# Autodesk Inventor assembly: Frame 1771926384246
(part 3 of 3)
212. ANSI UP8 x 30 - 125.591:133
213. ANSI UP8 x 30 - 125.591:134
214. ANSI UP8 x 30 - 125.591:135
215. ANSI UP8 x 30 - 81.102:79
216. ANSI UP8 x 30 - 125.591:136
217. ANSI UP8 x 30 - 125.591:137
218. ANSI UP8 x 30 - 125.591:138
219. ANSI UP8 x 30 - 81.102:80
220. ANSI UP8 x 30 - 125.591:139
221. ANSI UP8 x 30 - 125.591:140
222. ANSI UP8 x 30 - 81.102:81
223. ANSI UP8 x 30 - 125.591:141
224. ANSI UP8 x 30 - 125.591:142
225. ANSI UP8 x 30 - 81.102:82
226. ANSI UP8 x 30 - 125.591:143
227. ANSI UP8 x 30 - 81.102:83
228. ANSI UP8 x 30 - 125.591:144
229. ANSI UP8 x 30 - 125.591:145
230. ANSI UP8 x 30 - 125.591:146
231. ANSI UP8 x 30 - 125.591:147
232. ANSI UP8 x 30 - 81.102:84
233. ANSI UP8 x 30 - 125.591:148
234. ANSI UP8 x 30 - 125.591:149
235. ANSI UP8 x 30 - 81.102:85
236. ANSI UP8 x 30 - 81.102:86
237. ANSI UP8 x 30 - 125.591:150
238. ANSI UP8 x 30 - 125.591:151
239. ANSI UP8 x 30 - 81.102:87
240. ANSI UP8 x 30 - 125.591:152
241. ANSI UP8 x 30 - 81.102:88
242. ANSI UP8 x 30 - 125.591:153
243. ANSI UP8 x 30 - 81.102:89
244. ANSI UP8 x 30 - 125.591:154
245. ANSI UP8 x 30 - 81.102:90
246. ANSI UP8 x 30 - 125.591:155
247. ANSI UP8 x 30 - 81.102:91
248. ANSI UP8 x 30 - 81.102:92
249. ANSI UP8 x 30 - 125.591:156
250. ANSI UP8 x 30 - 125.591:157
251. ANSI UP8 x 30 - 81.102:93
252. ANSI UP8 x 30 - 81.102:94
253. ANSI UP8 x 30 - 125.591:158
254. ANSI UP8 x 30 - 125.591:159
255. ANSI UP8 x 30 - 81.102:95
256. ANSI UP8 x 30 - 81.102:96
257. ANSI UP8 x 30 - 125.591:160
258. ANSI UP8 x 30 - 125.591:161
259. ANSI UP8 x 30 - 81.102:97
260. ANSI UP8 x 30 - 81.102:98
261. ANSI UP8 x 30 - 125.591:162
262. ANSI UP8 x 30 - 125.591:163
263. ANSI UP8 x 30 - 125.591:164
264. ANSI UP8 x 30 - 125.591:165
265. ANSI UP8 x 30 - 125.591:166
266. ANSI UP8 x 30 - 125.591:167
267. ANSI UP8 x 30 - 125.591:168
268. ANSI UP8 x 30 - 125.591:169
269. ANSI UP8 x 30 - 125.591:170
270. ANSI UP8 x 30 - 125.591:171
271. ANSI UP8 x 30 - 125.591:172
272. ANSI UP8 x 30 - 125.591:173
273. ANSI UP8 x 30 - 125.591:174
274. ANSI UP8 x 30 - 125.591:175
275. ANSI UP8 x 30 - 81.102:99
276. ANSI UP8 x 30 - 81.102:100
277. ANSI UP8 x 30 - 125.591:176
278. ANSI UP8 x 30 - 125.591:177
279. ANSI UP8 x 30 - 125.591:178
280. ANSI UP8 x 30 - 125.591:179
281. ANSI UP8 x 30 - 81.102:101
282. ANSI UP8 x 30 - 125.591:180
283. ANSI UP8 x 30 - 125.591:181
284. ANSI UP8 x 30 - 81.102:102
285. ANSI UP8 x 30 - 125.591:182
286. ANSI UP8 x 30 - 125.591:183
287. ANSI UP8 x 30 - 81.102:103
288. ANSI UP8 x 30 - 125.591:184
289. ANSI UP8 x 30 - 81.102:104
290. ANSI UP8 x 30 - 125.591:185
291. ANSI UP8 x 30 - 125.591:186
292. ANSI UP8 x 30 - 81.102:105
293. ANSI UP8 x 30 - 125.591:187
294. ANSI UP8 x 30 - 125.591:188
295. ANSI UP8 x 30 - 81.102:106
296. ANSI UP8 x 30 - 125.591:189
297. ANSI UP8 x 30 - 81.102:107
298. ANSI UP8 x 30 - 125.591:190
299. ANSI UP8 x 30 - 81.102:108
300. ANSI UP8 x 30 - 125.591:191
301. ANSI UP8 x 30 - 81.102:109
302. ANSI UP8 x 30 - 125.591:192
303. ANSI UP8 x 30 - 81.102:110
304. ANSI UP8 x 30 - 125.591:193
305. ANSI UP8 x 30 - 81.102:111
306. ANSI UP8 x 30 - 125.591:194
307. ANSI UP8 x 30 - 81.102:112
308. ANSI UP8 x 30 - 125.591:195
309. ANSI UP8 x 30 - 81.102:113
310. ANSI UP8 x 30 - 125.591:196
311. ANSI UP8 x 30 - 81.102:114
312. ANSI UP8 x 30 - 125.591:197
313. ANSI UP8 x 30 - 81.102:115
314. ANSI UP8 x 30 - 81.102:116
315. ANSI UP8 x 30 - 125.591:198
316. ANSI UP8 x 30 - 125.591:199
317. ANSI UP8 x 30 - 81.102:117
318. ANSI UP8 x 30 - 81.102:118
319. ANSI UP8 x 30 - 125.591:200
320. ANSI UP8 x 30 - 125.591:201
321. ANSI UP8 x 30 - 81.102:119
322. ANSI UP8 x 30 - 81.102:120
323. ANSI UP8 x 30 - 125.591:202
324. ANSI UP8 x 30 - 125.591:203
325. ANSI UP8 x 30 - 125.591:204
326. ANSI UP8 x 30 - 125.591:205
327. ANSI UP8 x 30 - 125.591:206
328. ANSI UP8 x 30 - 125.591:207
329. ANSI UP8 x 30 - 125.591:208
330. ANSI UP8 x 30 - 125.591:209
331. ANSI UP8 x 30 - 125.591:210
332. ANSI UP8 x 30 - 125.591:211
333. ANSI UP8 x 30 - 125.591:212
334. ANSI UP8 x 30 - 125.591:213
335. ANSI UP8 x 30 - 125.591:214
336. ANSI UP8 x 30 - 125.591:215
337. ANSI UP8 x 30 - 125.591:216
338. ANSI UP8 x 30 - 81.102:121
339. ANSI UP8 x 30 - 125.591:217
340. ANSI UP8 x 30 - 125.591:218
341. ANSI UP8 x 30 - 81.102:122
342. ANSI UP8 x 30 - 125.591:219
343. ANSI UP8 x 30 - 125.591:220
344. ANSI UP8 x 30 - 81.102:123
345. ANSI UP8 x 30 - 81.102:124
346. ANSI UP8 x 30 - 125.591:221
347. ANSI UP8 x 30 - 125.591:222
348. ANSI UP8 x 30 - 125.591:223
349. ANSI UP8 x 30 - 125.591:224
350. ANSI UP8 x 30 - 81.102:125
351. ANSI UP8 x 30 - 125.591:225
352. ANSI UP8 x 30 - 125.591:226
353. ANSI UP8 x 30 - 81.102:126
354. ANSI UP8 x 30 - 125.591:227
355. ANSI UP8 x 30 - 125.591:228
356. ANSI UP8 x 30 - 125.591:229
357. ANSI UP8 x 30 - 125.591:230
358. ANSI UP8 x 30 - 81.102:127
359. ANSI UP8 x 30 - 81.102:128
360. ANSI UP8 x 30 - 125.591:231
361. ANSI UP8 x 30 - 81.102:129
362. ANSI UP8 x 30 - 125.591:232
363. ANSI UP8 x 30 - 81.102:130
364. ANSI UP8 x 30 - 81.102:131
365. ANSI UP8 x 30 - 125.591:233
366. ANSI UP8 x 30 - 125.591:234
367. ANSI UP8 x 30 - 81.102:132
368. ANSI UP8 x 30 - 125.591:235
369. ANSI UP8 x 30 - 125.591:236
370. ANSI UP8 x 30 - 81.102:133
371. ANSI UP8 x 30 - 81.102:134
372. ANSI UP8 x 30 - 125.591:237
373. ANSI UP8 x 30 - 81.102:135
374. ANSI UP8 x 30 - 125.591:238
375. ANSI UP8 x 30 - 125.591:239
376. ANSI UP8 x 30 - 81.102:136
377. ANSI UP8 x 30 - 81.102:137
378. ANSI UP8 x 30 - 125.591:240
379. ANSI UP8 x 30 - 81.102:138
380. ANSI UP8 x 30 - 81.102:139
381. ANSI UP8 x 30 - 125.591:241
382. ANSI UP8 x 30 - 125.591:242
383. ANSI UP8 x 30 - 81.102:140
384. ANSI UP8 x 30 - 125.591:243
385. ANSI UP8 x 30 - 125.591:244
386. ANSI UP8 x 30 - 81.102:141
387. ANSI UP8 x 30 - 125.591:245
388. ANSI UP8 x 30 - 125.591:246
389. ANSI UP8 x 30 - 125.591:247
390. ANSI UP8 x 30 - 125.591:248
391. ANSI UP8 x 30 - 125.591:249
392. ANSI UP8 x 30 - 125.591:250
393. ANSI UP8 x 30 - 125.591:251
394. ANSI UP8 x 30 - 125.591:252
395. ANSI UP8 x 30 - 125.591:253
396. ANSI UP8 x 30 - 125.591:254
397. ANSI UP8 x 30 - 125.591:255
398. ANSI UP8 x 30 - 125.591:256
399. ANSI UP8 x 30 - 125.591:257
400. ANSI UP8 x 30 - 125.591:258
401. ANSI UP8 x 30 - 81.102:142
402. ANSI UP8 x 30 - 125.591:259
403. ANSI UP8 x 30 - 81.102:143
404. ANSI UP8 x 30 - 125.591:260
405. ANSI UP8 x 30 - 125.591:261
406. ANSI UP8 x 30 - 81.102:144
407. ANSI UP8 x 30 - 125.591:262
408. ANSI UP8 x 30 - 125.591:263
409. ANSI UP8 x 30 - 125.591:264
410. ANSI UP8 x 30 - 81.102:145
411. ANSI UP8 x 30 - 125.591:265
412. ANSI UP8 x 30 - 125.591:266
413. ANSI UP8 x 30 - 81.102:146
414. ANSI UP8 x 30 - 125.591:267
415. ANSI UP8 x 30 - 125.591:268
416. ANSI UP8 x 30 - 81.102:147
417. ANSI UP8 x 30 - 81.102:148
418. ANSI UP8 x 30 - 125.591:269
419. ANSI UP8 x 30 - 125.591:270
420. ANSI UP8 x 30 - 125.591:271
421. ANSI UP8 x 30 - 125.591:272
422. ANSI UP8 x 30 - 125.591:273
423. ANSI UP8 x 30 - 81.102:149
424. ANSI UP8 x 30 - 81.102:150
425. ANSI UP8 x 30 - 81.102:151
426. ANSI UP8 x 30 - 125.591:274
427. ANSI UP8 x 30 - 125.591:275
428. ANSI UP8 x 30 - 81.102:152
429. ANSI UP8 x 30 - 81.102:153
430. ANSI UP8 x 30 - 125.591:276
431. ANSI UP8 x 30 - 125.591:277
432. ANSI UP8 x 30 - 81.102:154
433. ANSI UP8 x 30 - 125.591:278
434. ANSI UP8 x 30 - 81.102:155
435. ANSI UP8 x 30 - 125.591:279
436. ANSI UP8 x 30 - 81.102:156
437. ANSI UP8 x 30 - 81.102:157
438. ANSI UP8 x 30 - 125.591:280
439. ANSI UP8 x 30 - 81.102:158
440. ANSI UP8 x 30 - 125.591:281
441. ANSI UP8 x 30 - 81.102:159
442. ANSI UP8 x 30 - 125.591:282
443. ANSI UP8 x 30 - 81.102:160
444. ANSI UP8 x 30 - 125.591:283
445. ANSI UP8 x 30 - 125.591:284
446. ANSI UP8 x 30 - 81.102:161
447. ANSI UP8 x 30 - 125.591:285
448. ANSI UP8 x 30 - 81.102:162
449. ANSI UP8 x 30 - 81.102:163
450. ANSI UP8 x 30 - 125.591:286
451. ANSI UP8 x 30 - 81.102:164
452. ANSI UP8 x 30 - 125.591:287
453. ANSI UP8 x 30 - 125.591:288
454. ANSI UP8 x 30 - 125.591:289
455. ANSI UP8 x 30 - 125.591:290
456. ANSI UP8 x 30 - 125.591:291
457. ANSI UP8 x 30 - 125.591:292
458. ANSI UP8 x 30 - 125.591:293
459. ANSI UP8 x 30 - 125.591:294
460. ANSI UP8 x 30 - 125.591:295
461. ANSI UP8 x 30 - 125.591:296
462. ANSI UP8 x 30 - 125.591:297
463. ANSI UP8 x 30 - 125.591:298
464. ANSI UP8 x 30 - 125.591:299
465. ANSI UP8 x 30 - 125.591:300
466. ANSI UP8 x 30 - 125.591:301
467. ANSI UP8 x 30 - 125.591:302
468. ANSI UP8 x 30 - 81.102:165
469. ANSI UP8 x 30 - 125.591:303
470. ANSI UP8 x 30 - 125.591:304
471. ANSI UP8 x 30 - 81.102:166
472. ANSI UP8 x 30 - 125.591:305
473. ANSI UP8 x 30 - 81.102:167
474. ANSI UP8 x 30 - 125.591:306
475. ANSI UP8 x 30 - 81.102:168
476. ANSI UP8 x 30 - 125.591:307
477. ANSI UP8 x 30 - 125.591:308
478. ANSI UP8 x 30 - 125.591:309
479. ANSI UP8 x 30 - 81.102:169
480. ANSI UP8 x 30 - 125.591:310
481. ANSI UP8 x 30 - 81.102:170
482. ANSI UP8 x 30 - 125.591:311
483. ANSI UP8 x 30 - 125.591:312
484. ANSI UP8 x 30 - 125.591:313
485. ANSI UP8 x 30 - 81.102:171
486. ANSI UP8 x 30 - 81.102:172
487. ANSI UP8 x 30 - 125.591:314
488. ANSI UP8 x 30 - 125.591:315
489. ANSI UP8 x 30 - 81.102:173
490. ANSI UP8 x 30 - 125.591:316
491. ANSI UP8 x 30 - 125.591:317
492. ANSI UP8 x 30 - 81.102:174
493. ANSI UP8 x 30 - 81.102:175
494. ANSI UP8 x 30 - 125.591:318
495. ANSI UP8 x 30 - 81.102:176
496. ANSI UP8 x 30 - 125.591:319
497. ANSI UP8 x 30 - 81.102:177
498. ANSI UP8 x 30 - 125.591:320
499. ANSI UP8 x 30 - 81.102:178
500. ANSI UP8 x 30 - 125.591:321
501. ANSI UP8 x 30 - 81.102:179
502. ANSI UP8 x 30 - 81.102:180
503. ANSI UP8 x 30 - 125.591:322
504. ANSI UP8 x 30 - 125.591:323
505. ANSI UP8 x 30 - 125.591:324
506. ANSI UP8 x 30 - 81.102:181
507. ANSI UP8 x 30 - 81.102:182
508. ANSI UP8 x 30 - 125.591:325
509. ANSI UP8 x 30 - 125.591:326
510. ANSI UP8 x 30 - 125.591:327
511. ANSI UP8 x 30 - 81.102:183
512. ANSI UP8 x 30 - 81.102:184
513. ANSI UP8 x 30 - 81.102:185
514. ANSI UP8 x 30 - 81.102:186
515. ANSI UP8 x 30 - 125.591:328
516. ANSI UP8 x 30 - 125.591:329
517. ANSI UP8 x 30 - 125.591:330
518. ANSI UP8 x 30 - 125.591:331
519. ANSI UP8 x 30 - 125.591:332
520. ANSI UP8 x 30 - 125.591:333
521. ANSI UP8 x 30 - 125.591:334
522. ANSI UP8 x 30 - 125.591:335
523. ANSI UP8 x 30 - 125.591:336
524. ANSI UP8 x 30 - 125.591:337
525. ANSI UP8 x 30 - 125.591:338
526. ANSI UP8 x 30 - 125.591:339
527. ANSI UP8 x 30 - 125.591:340
528. ANSI UP8 x 30 - 125.591:341
529. ANSI UP8 x 30 - 125.591:342
530. ANSI UP8 x 30 - 125.591:343
531. ANSI UP8 x 30 - 81.102:187
532. ANSI UP8 x 30 - 125.591:344
533. ANSI UP8 x 30 - 81.102:188
534. ANSI UP8 x 30 - 125.591:345
535. ANSI UP8 x 30 - 125.591:346
536. ANSI UP8 x 30 - 125.591:347
537. ANSI UP8 x 30 - 81.102:189
538. ANSI UP8 x 30 - 125.591:348
539. ANSI UP8 x 30 - 81.102:190
540. ANSI UP8 x 30 - 125.591:349
541. ANSI UP8 x 30 - 125.591:350
542. ANSI UP8 x 30 - 125.591:351
543. ANSI UP8 x 30 - 125.591:352
544. ANSI UP8 x 30 - 81.102:191
545. ANSI UP8 x 30 - 125.591:353
546. ANSI UP8 x 30 - 125.591:354
547. ANSI UP8 x 30 - 81.102:192
548. ANSI UP8 x 30 - 81.102:193
549. ANSI UP8 x 30 - 125.591:355
550. ANSI UP8 x 30 - 81.102:194
551. ANSI UP8 x 30 - 125.591:356
552. ANSI UP8 x 30 - 81.102:195
553. ANSI UP8 x 30 - 81.102:196
554. ANSI UP8 x 30 - 81.102:197
555. ANSI UP8 x 30 - 125.591:357
556. ANSI UP8 x 30 - 125.591:358
557. ANSI UP8 x 30 - 125.591:359
558. ANSI UP8 x 30 - 81.102:198
559. ANSI UP8 x 30 - 81.102:199
560. ANSI UP8 x 30 - 125.591:360
561. ANSI UP8 x 30 - 81.102:200
562. ANSI UP8 x 30 - 81.102:201
563. ANSI UP8 x 30 - 125.591:361
564. ANSI UP8 x 30 - 125.591:362
565. ANSI UP8 x 30 - 81.102:202
566. ANSI UP8 x 30 - 81.102:203
567. ANSI UP8 x 30 - 125.591:363
568. ANSI UP8 x 30 - 125.591:364
569. ANSI UP8 x 30 - 125.591:365
570. ANSI UP8 x 30 - 81.102:204
571. ANSI UP8 x 30 - 81.102:205
572. ANSI UP8 x 30 - 125.591:366
573. ANSI UP8 x 30 - 125.591:367
574. ANSI UP8 x 30 - 81.102:206
575. ANSI UP8 x 30 - 81.102:207
576. ANSI UP8 x 30 - 125.591:368
577. ANSI UP8 x 30 - 125.591:369
578. ANSI UP8 x 30 - 125.591:370
579. ANSI UP8 x 30 - 125.591:371
580. ANSI UP8 x 30 - 125.591:372
581. ANSI UP8 x 30 - 125.591:373
582. ANSI UP8 x 30 - 125.591:374
583. ANSI UP8 x 30 - 125.591:375
584. ANSI UP8 x 30 - 125.591:376
585. ANSI UP8 x 30 - 125.591:377
586. ANSI UP8 x 30 - 125.591:378
587. ANSI UP8 x 30 - 125.591:379
588. ANSI UP8 x 30 - 125.591:380
589. ANSI UP8 x 30 - 81.102:208
590. ANSI UP8 x 30 - 125.591:381
591. ANSI UP8 x 30 - 125.591:382
592. ANSI UP8 x 30 - 81.102:209
593. ANSI UP8 x 30 - 125.591:383
594. ANSI UP8 x 30 - 125.591:384
595. ANSI UP8 x 30 - 81.102:210
596. ANSI UP8 x 30 - 125.591:385
597. ANSI UP8 x 30 - 81.102:211
598. ANSI UP8 x 30 - 125.591:386
599. ANSI UP8 x 30 - 125.591:387
600. ANSI UP8 x 30 - 81.102:212
601. ANSI UP8 x 30 - 125.591:388
602. ANSI UP8 x 30 - 125.591:389
603. ANSI UP8 x 30 - 125.591:390
604. ANSI UP8 x 30 - 81.102:213
605. ANSI UP8 x 30 - 125.591:391
606. ANSI UP8 x 30 - 125.591:392
607. ANSI UP8 x 30 - 81.102:214
608. ANSI UP8 x 30 - 81.102:215
609. ANSI UP8 x 30 - 81.102:216
610. ANSI UP8 x 30 - 125.591:393
611. ANSI UP8 x 30 - 81.102:217
612. ANSI UP8 x 30 - 81.102:218
613. ANSI UP8 x 30 - 125.591:394
614. ANSI UP8 x 30 - 125.591:395
615. ANSI UP8 x 30 - 81.102:219
616. ANSI UP8 x 30 - 125.591:396
617. ANSI UP8 x 30 - 81.102:220
618. ANSI UP8 x 30 - 125.591:397
619. ANSI UP8 x 30 - 81.102:221
620. ANSI UP8 x 30 - 81.102:222
621. ANSI UP8 x 30 - 125.591:398
622. ANSI UP8 x 30 - 125.591:399
623. ANSI UP8 x 30 - 81.102:223
624. ANSI UP8 x 30 - 125.591:400
625. ANSI UP8 x 30 - 125.591:401
626. ANSI UP8 x 30 - 81.102:224
627. ANSI UP8 x 30 - 81.102:225
628. ANSI UP8 x 30 - 81.102:226
629. ANSI UP8 x 30 - 125.591:402
630. ANSI UP8 x 30 - 125.591:403
631. ANSI UP8 x 30 - 125.591:404
632. ANSI UP8 x 30 - 125.591:405
633. ANSI UP8 x 30 - 125.591:406
634. ANSI UP8 x 30 - 125.591:407
635. ANSI UP8 x 30 - 125.591:408
636. ANSI UP8 x 30 - 125.591:409
637. ANSI UP8 x 30 - 125.591:410
638. ANSI UP8 x 30 - 125.591:411
639. ANSI UP8 x 30 - 125.591:412
640. ANSI UP8 x 30 - 125.591:413
641. ANSI UP8 x 30 - 125.591:414
642. ANSI UP8 x 30 - 81.102:227
643. ANSI UP8 x 30 - 125.591:415
644. ANSI UP8 x 30 - 125.591:416
645. ANSI UP8 x 30 - 81.102:228
646. ANSI UP8 x 30 - 125.591:417
647. ANSI UP8 x 30 - 125.591:418
648. ANSI UP8 x 30 - 81.102:229
649. ANSI UP8 x 30 - 125.591:419
650. ANSI UP8 x 30 - 81.102:230
651. ANSI UP8 x 30 - 125.591:420
652. ANSI UP8 x 30 - 125.591:421
653. ANSI UP8 x 30 - 125.591:422
654. ANSI UP8 x 30 - 125.591:423
655. ANSI UP8 x 30 - 81.102:231
656. ANSI UP8 x 30 - 81.102:232
657. ANSI UP8 x 30 - 125.591:424
658. ANSI UP8 x 30 - 81.102:233
659. ANSI UP8 x 30 - 81.102:234
660. ANSI UP8 x 30 - 125.591:425
661. ANSI UP8 x 30 - 81.102:235
662. ANSI UP8 x 30 - 81.102:236
663. ANSI UP8 x 30 - 125.591:426
664. ANSI UP8 x 30 - 125.591:427
665. ANSI UP8 x 30 - 81.102:237
666. ANSI UP8 x 30 - 125.591:428
667. ANSI UP8 x 30 - 81.102:238
668. ANSI UP8 x 30 - 125.591:429
669. ANSI UP8 x 30 - 81.102:239
670. ANSI UP8 x 30 - 81.102:240
671. ANSI UP8 x 30 - 125.591:430
672. ANSI UP8 x 30 - 125.591:431
673. ANSI UP8 x 30 - 81.102:241
674. ANSI UP8 x 30 - 125.591:432
675. ANSI UP8 x 30 - 81.102:242
676. ANSI UP8 x 30 - 125.591:433
677. ANSI UP8 x 30 - 125.591:434
678. ANSI UP8 x 30 - 125.591:435
679. ANSI UP8 x 30 - 125.591:436
680. ANSI UP8 x 30 - 125.591:437
681. ANSI UP8 x 30 - 125.591:438
682. ANSI UP8 x 30 - 125.591:439
683. ANSI UP8 x 30 - 125.591:440
684. ANSI UP8 x 30 - 125.591:441
685. ANSI UP8 x 30 - 125.591:442
686. ANSI UP8 x 30 - 81.102:243
687. ANSI UP8 x 30 - 125.591:443
688. ANSI UP8 x 30 - 125.591:444
689. ANSI UP8 x 30 - 81.102:244
690. ANSI UP8 x 30 - 125.591:445
691. ANSI UP8 x 30 - 125.591:446
692. ANSI UP8 x 30 - 81.102:245
693. ANSI UP8 x 30 - 125.591:447
694. ANSI UP8 x 30 - 125.591:448
695. ANSI UP8 x 30 - 125.591:449
696. ANSI UP8 x 30 - 81.102:246
697. ANSI UP8 x 30 - 125.591:450
698. ANSI UP8 x 30 - 81.102:247
699. ANSI UP8 x 30 - 81.102:248
700. ANSI UP8 x 30 - 125.591:451
701. ANSI UP8 x 30 - 81.102:249
702. ANSI UP8 x 30 - 81.102:250
703. ANSI UP8 x 30 - 81.102:251
704. ANSI UP8 x 30 - 125.591:452
705. ANSI UP8 x 30 - 125.591:453
706. ANSI UP8 x 30 - 81.102:252
707. ANSI UP8 x 30 - 125.591:454
708. ANSI UP8 x 30 - 81.102:253
709. ANSI UP8 x 30 - 125.591:455
710. ANSI UP8 x 30 - 81.102:254
711. ANSI UP8 x 30 - 81.102:255
712. ANSI UP8 x 30 - 125.591:456
713. ANSI UP8 x 30 - 125.591:457
714. ANSI UP8 x 30 - 125.591:458
715. ANSI UP8 x 30 - 125.591:459
716. ANSI UP8 x 30 - 125.591:460
717. ANSI UP8 x 30 - 125.591:461
718. ANSI UP8 x 30 - 125.591:462
719. ANSI UP8 x 30 - 125.591:463
720. ANSI UP8 x 30 - 125.591:464
721. ANSI UP8 x 30 - 81.102:256
722. ANSI UP8 x 30 - 125.591:465
723. ANSI UP8 x 30 - 81.102:257
724. ANSI UP8 x 30 - 125.591:466
725. ANSI UP8 x 30 - 125.591:467
726. ANSI UP8 x 30 - 81.102:258
727. ANSI UP8 x 30 - 125.591:468
728. ANSI UP8 x 30 - 125.591:469
729. ANSI UP8 x 30 - 125.591:470
730. ANSI UP8 x 30 - 81.102:259
731. ANSI UP8 x 30 - 81.102:260
732. ANSI UP8 x 30 - 81.102:261
733. ANSI UP8 x 30 - 125.591:471
734. ANSI UP8 x 30 - 81.102:262
735. ANSI UP8 x 30 - 125.591:472
736. ANSI UP8 x 30 - 125.591:473
737. ANSI UP8 x 30 - 81.102:263
738. ANSI UP8 x 30 - 81.102:264
739. ANSI UP8 x 30 - 125.591:474
740. ANSI UP8 x 30 - 81.102:265
741. ANSI UP8 x 30 - 125.591:475
742. ANSI UP8 x 30 - 125.591:476
743. ANSI UP8 x 30 - 125.591:477
744. ANSI UP8 x 30 - 125.591:478
745. ANSI UP8 x 30 - 125.591:479
746. ANSI UP8 x 30 - 125.591:480
747. ANSI UP8 x 30 - 81.102:266
748. ANSI UP8 x 30 - 125.591:481
749. ANSI UP8 x 30 - 81.102:267
750. ANSI UP8 x 30 - 125.591:482
751. ANSI UP8 x 30 - 125.591:483
752. ANSI UP8 x 30 - 81.102:268
753. ANSI UP8 x 30 - 125.591:484
754. ANSI UP8 x 30 - 81.102:269
755. ANSI UP8 x 30 - 125.591:485
756. ANSI UP8 x 30 - 81.102:270
757. ANSI UP8 x 30 - 81.102:271
758. ANSI UP8 x 30 - 125.591:486
759. ANSI UP8 x 30 - 81.102:272
760. ANSI UP8 x 30 - 125.591:487
761. ANSI UP8 x 30 - 125.591:488
762. ANSI UP8 x 30 - 125.591:489
763. ANSI UP8 x 30 - 125.591:490
764. ANSI UP8 x 30 - 125.591:491
765. ANSI UP8 x 30 - 81.102:273
766. ANSI UP8 x 30 - 81.102:274
767. ANSI UP8 x 30 - 125.591:492
768. ANSI UP8 x 30 - 81.102:275
769. ANSI UP8 x 30 - 81.102:276
770. ANSI UP8 x 30 - 125.591:493
771. ANSI UP8 x 30 - 125.591:494
772. ANSI UP8 x 30 - 81.102:277
773. ANSI UP8 x 30 - 125.591:495
774. ANSI UP8 x 30 - 81.102:278
775. ANSI UP8 x 30 - 81.102:279
776. ANSI UP8 x 30 - 125.591:496
777. ANSI UP8 x 30 - 125.591:497
778. ANSI UP8 x 30 - 81.102:280
779. ANSI UP8 x 30 - 125.591:498
780. ANSI UP8 x 30 - 125.591:499
781. ANSI UP8 x 30 - 125.591:500
782. ANSI UP8 x 30 - 81.102:281
783. ANSI UP8 x 30 - 125.591:501
784. ANSI UP8 x 30 - 81.102:282
785. ANSI UP8 x 30 - 125.591:502
786. ANSI UP8 x 30 - 125.591:503
787. ANSI UP8 x 30 - 125.591:504
788. ANSI UP8 x 30 - 125.591:505
789. ANSI UP8 x 30 - 125.591:506
790. ANSI UP8 x 30 - 81.102:283
791. ANSI UP8 x 30 - 125.591:507
792. ANSI UP8 x 30 - 125.591:508
793. ANSI UP8 x 30 - 81.102:284
794. ANSI UP8 x 30 - 81.102:285
795. ANSI UP8 x 30 - 125.591:509
796. ANSI UP8 x 30 - 125.591:510
797. ANSI UP8 x 30 - 81.102:286
798. ANSI UP8 x 30 - 125.591:511
799. ANSI UP8 x 30 - 125.591:512
800. ANSI UP8 x 30 - 125.591:513
801. ANSI UP8 x 30 - 125.591:514
802. ANSI UP8 x 30 - 81.102:287
803. ANSI UP8 x 30 - 125.591:515
804. ANSI UP8 x 30 - 125.591:516
805. ANSI UP8 x 30 - 81.102:288
806. ANSI UP8 x 30 - 125.591:517
807. ANSI UP8 x 30 - 125.591:518
808. ANSI UP8 x 30 - 125.591:519
809. ANSI UP8 x 30 - 81.102:289
810. ANSI UP8 x 30 - 125.591:520
811. ANSI UP8 x 30 - 125.591:521
812. ANSI UP8 x 30 - 81.102:290
813. ANSI UP8 x 30 - 125.591:522
814. ANSI UP8 x 30 - 125.591:523
815. ANSI UP8 x 30 - 125.591:524
816. ANSI UP8 x 30 - 125.591:525
817. ANSI UP8 x 30 - 81.102:291
818. ANSI UP8 x 30 - 125.591:526
819. ANSI UP8 x 30 - 125.591:527
820. ANSI UP8 x 30 - 125.591:528
821. ANSI UP8 x 30 - 125.591:529
822. ANSI UP8 x 30 - 81.102:292
823. ANSI UP8 x 30 - 81.102:293
824. ANSI UP8 x 30 - 125.591:530
825. ANSI UP8 x 30 - 125.591:531
826. ANSI UP8 x 30 - 125.591:532
827. ANSI UP8 x 30 - 125.591:533
828. ANSI UP8 x 30 - 125.591:534
829. ANSI UP8 x 30 - 125.591:535
830. ANSI UP8 x 30 - 81.102:294
831. ANSI UP8 x 30 - 81.102:295
832. ANSI UP8 x 30 - 81.102:296
833. ANSI UP8 x 30 - 125.591:536
834. ANSI UP8 x 30 - 125.591:537
835. ANSI UP8 x 30 - 125.591:538
836. ANSI UP8 x 30 - 81.102:297
837. ANSI UP8 x 30 - 125.591:539
838. ANSI UP8 x 30 - 125.591:540
839. ANSI UP8 x 30 - 81.102:298
840. ANSI UP8 x 30 - 81.102:299
841. ANSI UP8 x 30 - 81.102:300
